# Autodesk Inventor assembly: 6inchMiniCimShooter_MIR1
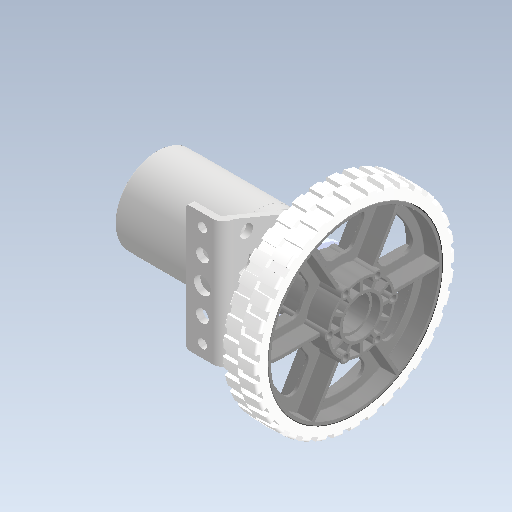
[picture p0: Inventor's stored thumbnail of the model, 512x512]
Saved by Autodesk Inventor 2020.2 (Build 242310000, 310)
## iProperties
Created: 2020-01-18
Part Number: 6inchMiniCimShooter_MIR1
Document SubType Name: Assembly
Designer: robst
Author: robst
## Documents named in this file (5)
- C:\git\CAD-Development\robSteele\2020BallTriggerMechanism\6inchMiniCimShooter_MIR1.iam
- C:\git\CAD-Development\robSteele\2020BallTriggerMechanism\AM 2488 CIM bracket_MIR1.ipt
- C:\git\CAD-Development\robSteele\2020BallTriggerMechanism\Mini_CIM_Motor_217-3371_MIR1.ipt
- C:\git\CAD-Development\robSteele\2020BallTriggerMechanism\am-0320a_8mm_Key_Hub_MIR1.ipt
- C:\git\CAD-Development\robSteele\2020BallTriggerMechanism\am-940a-6-HiGrip-_MIR1.iam
## Components (4 placed, 4 different names)
1. AM 2488 CIM bracket_MIR1:1 — Insert:2, Insert:1
2. Mini_CIM_Motor_217-3371_MIR1:1 — Insert:2, Insert:1, Insert:3
3. am-0320a_8mm_Key_Hub_MIR1:1 — Insert:3, Insert:4
4. am-940a-6-HiGrip-_MIR1:1 [sub-assembly] — Insert:4
## Relationships (4: Insert 4)
- Insert:2: AM 2488 CIM bracket_MIR1:1 ↔ Mini_CIM_Motor_217-3371_MIR1:1
- Insert:1: AM 2488 CIM bracket_MIR1:1 ↔ Mini_CIM_Motor_217-3371_MIR1:1
- Insert:3: Mini_CIM_Motor_217-3371_MIR1:1 ↔ am-0320a_8mm_Key_Hub_MIR1:1
- Insert:4: am-0320a_8mm_Key_Hub_MIR1:1 ↔ am-940a-6-HiGrip-_MIR1:1
